# Autodesk Inventor assembly: X-axis Motor Assembly
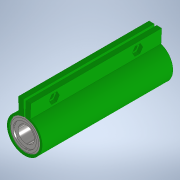
[picture p0: Inventor's stored thumbnail of the model, 180x180]
Saved by Autodesk Inventor 2020 (Build 240168000, 168)
## iProperties
Created: 2019-09-15
Part Number: X-axis Motor Assembly
Document SubType Name: Assembly
Designer: pepd9
Author: pepd9
## Documents named in this file (3)
- C:\DESIGNS\MK3PRO BOWDEN\X-axis Motor Assembly.iam
- C:\DESIGNS\MK3PRO BOWDEN\X-Motor P1.ipt
- C:\DESIGNS\MK3PRO BOWDEN\LM10UU.ipt
## Components (3 placed, 2 different names)
1. X-Motor P1:1 — Mate:1, Mate:2, Flush:1, Flush:2
2. LM10UU:1 — Mate:1, Flush:2
3. LM10UU:2 — Mate:2, Flush:1
## Relationships (4: Mate 2, Flush 2)
- Mate:1: X-Motor P1:1 ↔ LM10UU:1
- Mate:2: X-Motor P1:1 ↔ LM10UU:2
- Flush:1: X-Motor P1:1 ↔ LM10UU:2
- Flush:2: X-Motor P1:1 ↔ LM10UU:1
